# Autodesk Inventor assembly: AXp2p
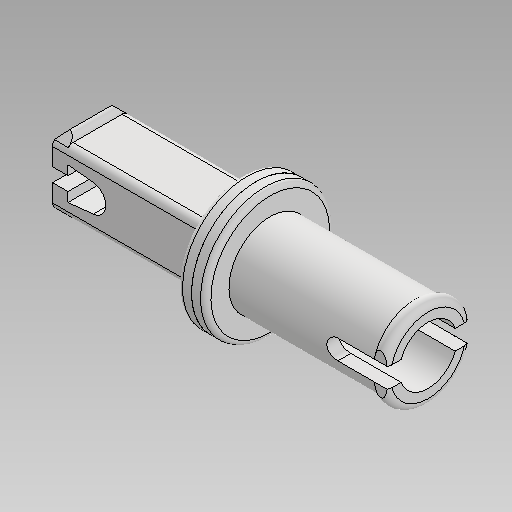
[picture p0: Inventor's stored thumbnail of the model, 512x512]
Saved by Autodesk Inventor 2020 (Build 240168000, 168)
## iProperties
Created: 2019-05-09
Part Number: AXp2p
Document SubType Name: Assembly
Designer: Varga Daniel
Author: Varga Daniel
## Documents named in this file (4)
- C:\!_Dani\!_cloud\OneDrive\!_munka\Revolution\StructuralParts\Axles\AXpXp\AXp2p_no_anti_skid.iam
- C:\!_Dani\!_cloud\OneDrive\!_munka\Revolution\StructuralParts\Connector pins\Connector_pin_base_square.ipt
- C:\!_Dani\!_cloud\OneDrive\!_munka\Revolution\StructuralParts\Connector pins\Connector_pin_base\Connector_pin_base_single_no_anti_skid.ipt
- C:\!_Dani\!_cloud\OneDrive\!_munka\Revolution\StructuralParts\Connector pins\Connector_pin_base.ipt
## Components (2 placed, 2 different names)
1. Connector_pin_base_square:1 — Mate:1, Mate:2, Flush:1
2. Connector_pin_base_single_no_anti_skid:1 — Mate:3, Mate:4, Flush:2
## Relationships (6: Mate 4, Flush 2)
- Mate:1: Connector_pin_base_square:1
- Mate:2: Connector_pin_base_square:1
- Flush:1: Connector_pin_base_square:1
- Mate:3: Connector_pin_base_single_no_anti_skid:1
- Mate:4: Connector_pin_base_single_no_anti_skid:1
- Flush:2: Connector_pin_base_single_no_anti_skid:1
